# Autodesk Inventor assembly: BandSawJigAssembly
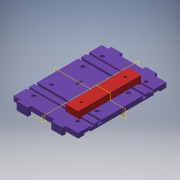
[picture p0: Inventor's stored thumbnail of the model, 180x180]
Saved by Autodesk Inventor 2018.2 (Build 222227000, 227)
## iProperties
Created: 2017-12-10
Part Number: BandSawJigAssembly
Document SubType Name: Assembly
Designer: steele
Author: steele
## Documents named in this file (4)
- D:\snobotics\CAD-Development\robSteele\HouseProjects\Garage\BandSawJigAssembly.iam
- D:\snobotics\CAD-Development\robSteele\HouseProjects\Garage\BandSawJigBottom.ipt
- D:\snobotics\CAD-Development\robSteele\HouseProjects\Garage\BandSawJigTop.ipt
- D:\snobotics\CAD-Development\robSteele\HouseProjects\Garage\BandSawJigSupport.ipt
## Components (3 placed, 3 different names)
1. BandSawJigBottom:1 — Mate:1, Flush:1, Mate:2, Mate:3
2. BandSawJigTop:1 — Mate:1, Flush:1
3. BandSawJigSupport:1 — Mate:2, Mate:3
## Relationships (4: Mate 3, Flush 1)
- Mate:1: BandSawJigBottom:1 ↔ BandSawJigTop:1
- Flush:1 (-50.8 mm): BandSawJigBottom:1 ↔ BandSawJigTop:1
- Mate:2: BandSawJigBottom:1 ↔ BandSawJigSupport:1
- Mate:3: BandSawJigBottom:1 ↔ BandSawJigSupport:1
